# Autodesk Inventor assembly: s-assy-scara-unit-j2_sub
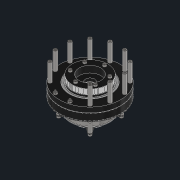
[picture p0: Inventor's stored thumbnail of the model, 180x180]
Saved by Autodesk Inventor 2022 (Build 260153000, 153)
## iProperties
Created: 2021-07-12
Document SubType Name: Assembly
Designer: yuta0
Mass: 2750.98 g
Surface Area: 6960.57 cm^2
Volume: 1238.47 cm^3
Density: 2.22127 g/cm^3
Part Number: s-assy-scara-unit-j2_sub
Author: yuta0
## Documents named in this file (9)
- C:\Users\yuta0\Desktop\assy-scara\s-assy-scara-unit-j2_sub.iam
- C:\Users\yuta0\Desktop\assy-scara\s-assy-sun_gear.iam
- C:\Users\yuta0\Desktop\assy-scara\s-assy-unit-j2-2-gear.iam
- C:\Users\yuta0\Desktop\assy-scara\scara-base2.ipt
- C:\Users\yuta0\Desktop\assy-scara\s-assy-ring_gear-2.iam
- C:\Users\yuta0\Desktop\assy-scara\CB4-35.ipt
- C:\Users\yuta0\Desktop\assy-scara\ARF-440E.ipt
- C:\Users\yuta0\Desktop\assy-scara\LBNR4.ipt
- C:\Users\yuta0\Documents\GitHub\catchrobo_hardware\assy-robot\s-assy-unit-j3.iam
## Components (34 placed, 7 different names)
1. s-assy-sun_gear:1 [sub-assembly] — メイト:1, メイト:2, メイト:70
2. s-assy-unit-j2-2-gear:1 [sub-assembly] — メイト:1, フラッシュ:1, メイト:2, メイト:52, メイト:53, メイト:69, メイト:71, メイト:72, メイト:93
3. s-assy-ring_gear-2:1 [sub-assembly] — メイト:52, メイト:53, メイト:70, メイト:115, メイト:116, メイト:117, メイト:118, メイト:119, メイト:120, メイト:122
4. scara-base2:1 — メイト:69, メイト:71, メイト:72, メイト:93, メイト:113, メイト:114
5. CB4-35:2 — メイト:113, メイト:114
6. CB4-35:3
7. CB4-35:4
8. CB4-35:5
9. CB4-35:6
10. CB4-35:7
11. ARF-440E:1 — メイト:115, メイト:116
12. CB4-35:8 — メイト:117, メイト:118
13. ARF-440E:2
14. CB4-35:9
15. ARF-440E:3
16. CB4-35:10
17. ARF-440E:4
18. CB4-35:11
19. ARF-440E:5
20. CB4-35:12
21. ARF-440E:6
22. CB4-35:13
23. ARF-440E:7
24. CB4-35:14
25. ARF-440E:8
26. CB4-35:15
27. ARF-440E:9
28. CB4-35:16
29. ARF-440E:10
30. CB4-35:17
31. CB4-35:18 — メイト:119, メイト:120, メイト:121
32. LBNR4:1 — メイト:121, メイト:122
33. CB4-35:19
34. LBNR4:2
## Component patterns: (6 elements, first: CB4-35:2), (10 elements, first: ARF-440E:1 + CB4-35:8), (2 elements, first: CB4-35:18 + LBNR4:1)
## Relationships (20: Mate 19, Flush 1)
- メイト:1 [Mate]: s-assy-sun_gear:1 ↔ s-assy-unit-j2-2-gear:1
- フラッシュ:1 [Flush]: s-assy-unit-j2-2-gear:1
- メイト:2 [Mate]: s-assy-sun_gear:1 ↔ s-assy-unit-j2-2-gear:1
- メイト:52 [Mate]: s-assy-unit-j2-2-gear:1 ↔ s-assy-ring_gear-2:1
- メイト:53 [Mate]: s-assy-unit-j2-2-gear:1 ↔ s-assy-ring_gear-2:1
- メイト:69 [Mate]: s-assy-unit-j2-2-gear:1 ↔ scara-base2:1
- メイト:70 [Mate]: s-assy-sun_gear:1 ↔ s-assy-ring_gear-2:1
- メイト:71 [Mate]: s-assy-unit-j2-2-gear:1 ↔ scara-base2:1
- メイト:72 [Mate]: s-assy-unit-j2-2-gear:1 ↔ scara-base2:1
- メイト:93 [Mate]: s-assy-unit-j2-2-gear:1 ↔ scara-base2:1
- メイト:113 [Mate]: scara-base2:1 ↔ CB4-35:2
- メイト:114 [Mate]: scara-base2:1 ↔ CB4-35:2
- メイト:115 [Mate]: s-assy-ring_gear-2:1 ↔ ARF-440E:1
- メイト:116 [Mate]: s-assy-ring_gear-2:1 ↔ ARF-440E:1
- メイト:117 [Mate]: s-assy-ring_gear-2:1 ↔ CB4-35:8
- メイト:118 [Mate]: s-assy-ring_gear-2:1 ↔ CB4-35:8
- メイト:119 [Mate]: s-assy-ring_gear-2:1 ↔ CB4-35:18
- メイト:120 [Mate]: s-assy-ring_gear-2:1 ↔ CB4-35:18
- メイト:121 [Mate]: CB4-35:18 ↔ LBNR4:1
- メイト:122 [Mate]: s-assy-ring_gear-2:1 ↔ LBNR4:1
